# Autodesk Inventor assembly: fullPCIshortconnector
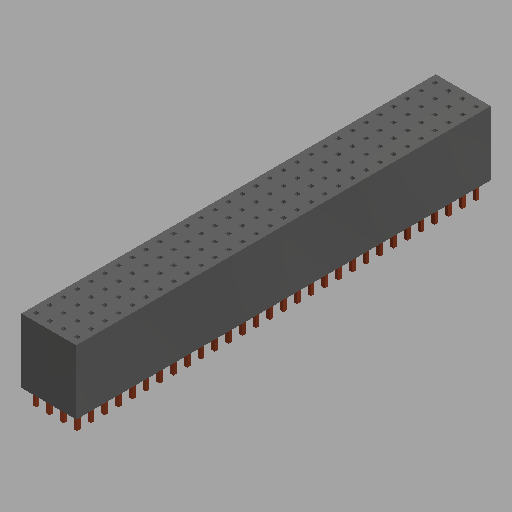
[picture p0: Inventor's stored thumbnail of the model, 512x512]
Saved by Autodesk Inventor 2022 (Build 260153000, 153)
## iProperties
Created: 2021-10-08
Part Number: fullPCIshortconnector
Document SubType Name: Assembly
Designer: Bowen O'Steen
Author: Bowen O'Steen
## Documents named in this file (3)
- C:\Users\gwhen\OneDrive\Desktop\Vault\Designs\MEMESat\MemeSat\Engineering Data\MemeSat\Subsystems\fullPCIshortconnector.iam
- C:\Users\gwhen\OneDrive\Desktop\Vault\Designs\MEMESat\MemeSat\Engineering Data\MemeSat\Subsystems\PCIconnector.ipt
- C:\Users\gwhen\OneDrive\Desktop\Vault\Designs\MEMESat\MemeSat\Engineering Data\MemeSat\Subsystems\PCIshortpins.ipt
## Components (2 placed, 2 different names)
1. PCIconnector:1 — Flush:1, Flush:2, Flush:3, Mate:1, Mate:2, Mate:3
2. PCIshortpins:1 — Mate:1, Mate:2, Mate:3
## Relationships (6: Flush 3, Mate 3)
- Flush:1: PCIconnector:1
- Flush:2: PCIconnector:1
- Flush:3: PCIconnector:1
- Mate:1: PCIconnector:1 ↔ PCIshortpins:1
- Mate:2: PCIconnector:1 ↔ PCIshortpins:1
- Mate:3 (-4.59 mm): PCIconnector:1 ↔ PCIshortpins:1
